# Autodesk Inventor assembly: Assembly2
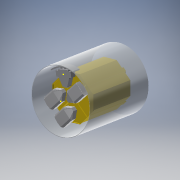
[picture p0: Inventor's stored thumbnail of the model, 180x180]
Saved by Autodesk Inventor 2018 (Build 220112000, 112)
## iProperties
Created: 2021-03-15
Part Number: Assembly2
Document SubType Name: Assembly
Designer: dell
Author: dell
## Documents named in this file (4)
- D:\Autodesk\Projects\C-C\a1\ES101 GROUP-13 PROJECT\FINAL MODEL\Resolved files\Assembly2.iam
- D:\Autodesk\Projects\C-C\a1\ES101 GROUP-13 PROJECT\FINAL MODEL\Resolved files\Assembly1.iam
- D:\Autodesk\Projects\C-C\a1\ES101 GROUP-13 PROJECT\INDIVIDUAL WORK\Keval\Aft shroud.ipt
- D:\Autodesk\Projects\C-C\a1\ES101 GROUP-13 PROJECT\INDIVIDUAL WORK\Keval\Resolved files\Derived WFC3(part1).ipt
## Components (3 placed, 3 different names)
1. Assembly1:1 [sub-assembly] — Mate:3, Mate:4, Flush:1, Mate:5, Mate:6
2. Aft shroud:1 — Mate:3
3. Derived WFC3(part1):1 — Mate:4, Flush:1, Mate:5, Mate:6
## Relationships (5: Mate 4, Flush 1)
- Mate:3: Assembly1:1 ↔ Aft shroud:1
- Mate:4 (10 mm): Assembly1:1 ↔ Derived WFC3(part1):1
- Flush:1: Assembly1:1 ↔ Derived WFC3(part1):1
- Mate:5 (20 mm): Assembly1:1 ↔ Derived WFC3(part1):1
- Mate:6 (26 mm): Assembly1:1 ↔ Derived WFC3(part1):1
